# Autodesk Inventor assembly: AM14U3 Long Half
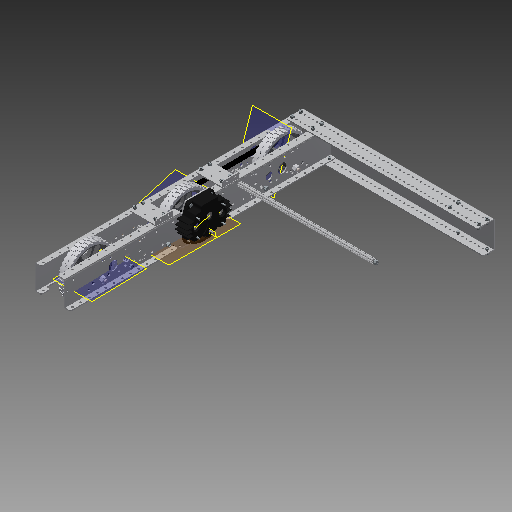
[picture p0: Inventor's stored thumbnail of the model, 512x512]
Saved by Autodesk Inventor 2018 (Build 220112000, 112)
## iProperties
Created: 2015-12-05
Part Number: AM14U3 Long Half
Document SubType Name: Assembly
Designer: PhillipD
Author: PhillipD
Revision Number: ANY
## Documents named in this file (9)
- D:\FIRST 2018\FIRST 2018 Inventor\FIRST 2017 Drive Base\Parts\AM14U3 Long Half.iam
- D:\FIRST 2018\FIRST 2018 Inventor\FIRST 2017 Drive Base\Parts\AM14U3 Long Frame Half.iam
- D:\FIRST 2018\FIRST 2018 Inventor\FIRST 2017 Drive Base\Parts\6 HiGrip with bearings, pulleys and spacers.iam
- D:\FIRST 2018\FIRST 2018 Inventor\FIRST 2017 Drive Base\Parts\6 HiGrip with hub and double pulley.iam
- D:\FIRST 2018\FIRST 2018 Inventor\FIRST 2017 Drive Base\Parts\am-2598_107 2016 KOP Toughbox Mini.iam
- D:\FIRST 2018\FIRST 2018 Inventor\FIRST 2017 Drive Base\Parts\FR8ZZ Hex Bearing.ipt
- D:\FIRST 2018\FIRST 2018 Inventor\FIRST 2017 Drive Base\Parts\am-2266 800-5M-15 v2 Timing Belt.ipt
- D:\FIRST 2018\FIRST 2018 Inventor\FIRST 2017 Drive Base\Parts\375-16 x 4.25 Hex Bolt_HFBOLT 0.375-16x2.5x1-C.ipt
- D:\FIRST 2018\FIRST 2018 Inventor\FIRST 2017 Drive Base\Parts\375-16 Lock Nut_91831A127.ipt
## Components (12 placed, 12 different names)
1. AM14U3 Long Frame Half_3 [sub-assembly] — Insert:1, Angle:1, Insert:2, Angle:2, Insert:3, Insert:4, Angle:3, Insert:5, Insert:6, Insert:7, Insert:9, Insert:10
2. 6 HiGrip with bearings, pulleys and spacers_4 [sub-assembly] — Insert:3
3. 6 HiGrip with bearings, pulleys and spacers_5 [sub-assembly] — Insert:6
4. 6 HiGrip with hub and double pulley_6 [sub-assembly] — Insert:8, Angle:4, Angle:5, Angle:7, Mate:1
5. am-2598_107 2016 KOP Toughbox Mini_7 [sub-assembly] — Insert:9, Insert:10, Angle:5, Angle:6, Angle:7
6. FR8ZZ Hex Bearing_8 — Insert:7, Insert:8, Angle:4, Angle:6
7. am-2266 800-5M-15 v2 Timing Belt_9 — Mate:2
8. am-2266 800-5M-15 v2 Timing Belt_10 — Mate:1
9. 375-16 x 4.25 Hex Bolt_HFBOLT 0.375-16x2.5x1-C_11 — Insert:1, Angle:1, Mate:2
10. 375-16 x 4.25 Hex Bolt_HFBOLT 0.375-16x2.5x1-C_12 — Insert:4, Angle:3
11. 375-16 Lock Nut_91831A127_13 — Insert:5
12. 375-16 Lock Nut_91831A127_14 — Insert:2, Angle:2
## Relationships (19: Insert 10, Angle 7, Mate 2)
- Insert:1: AM14U3 Long Frame Half_3 ↔ 375-16 x 4.25 Hex Bolt_HFBOLT 0.375-16x2.5x1-C_11
- Angle:1 (0 deg): AM14U3 Long Frame Half_3 ↔ 375-16 x 4.25 Hex Bolt_HFBOLT 0.375-16x2.5x1-C_11
- Insert:2: AM14U3 Long Frame Half_3 ↔ 375-16 Lock Nut_91831A127_14
- Angle:2 (0 deg): AM14U3 Long Frame Half_3 ↔ 375-16 Lock Nut_91831A127_14
- Insert:3 (0.0762 mm): AM14U3 Long Frame Half_3 ↔ 6 HiGrip with bearings, pulleys and spacers_4
- Insert:4: AM14U3 Long Frame Half_3 ↔ 375-16 x 4.25 Hex Bolt_HFBOLT 0.375-16x2.5x1-C_12
- Angle:3 (0 deg): AM14U3 Long Frame Half_3 ↔ 375-16 x 4.25 Hex Bolt_HFBOLT 0.375-16x2.5x1-C_12
- Insert:5: AM14U3 Long Frame Half_3 ↔ 375-16 Lock Nut_91831A127_13
- Insert:6 (0.0762 mm): AM14U3 Long Frame Half_3 ↔ 6 HiGrip with bearings, pulleys and spacers_5
- Insert:7: AM14U3 Long Frame Half_3 ↔ FR8ZZ Hex Bearing_8
- Insert:8: 6 HiGrip with hub and double pulley_6 ↔ FR8ZZ Hex Bearing_8
- Angle:4 (10 deg): 6 HiGrip with hub and double pulley_6 ↔ FR8ZZ Hex Bearing_8
- Insert:9: AM14U3 Long Frame Half_3 ↔ am-2598_107 2016 KOP Toughbox Mini_7
- Insert:10: AM14U3 Long Frame Half_3 ↔ am-2598_107 2016 KOP Toughbox Mini_7
- Angle:5 (0 deg): 6 HiGrip with hub and double pulley_6 ↔ am-2598_107 2016 KOP Toughbox Mini_7
- Angle:6 (0 deg): am-2598_107 2016 KOP Toughbox Mini_7 ↔ FR8ZZ Hex Bearing_8
- Angle:7 (0 deg): 6 HiGrip with hub and double pulley_6 ↔ am-2598_107 2016 KOP Toughbox Mini_7
- Mate:1: 6 HiGrip with hub and double pulley_6 ↔ am-2266 800-5M-15 v2 Timing Belt_10
- Mate:2: am-2266 800-5M-15 v2 Timing Belt_9 ↔ 375-16 x 4.25 Hex Bolt_HFBOLT 0.375-16x2.5x1-C_11
